# Autodesk Inventor assembly: DIFF_HOUSING_FINAL_ASM
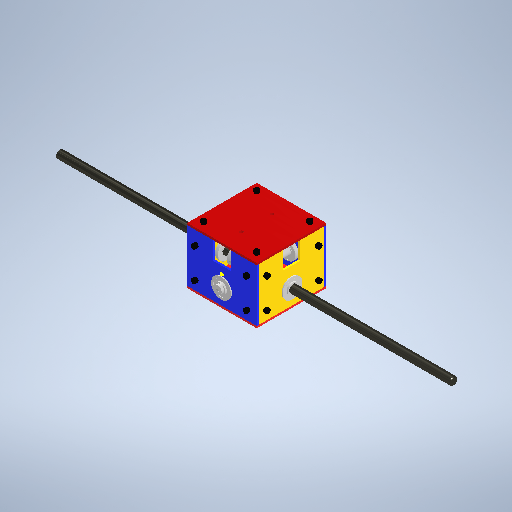
[picture p0: Inventor's stored thumbnail of the model, 512x512]
Saved by Autodesk Inventor 2025.1 (Build 291241000, 241)
## iProperties
Created: 2023-11-30
Part Number: DIFF_HOUSING_FINAL_ASM
Document SubType Name: Assembly
Designer: bugme
Author: bugme
## Documents named in this file (10)
- C:\Users\bugme\OneDrive - The Pennsylvania State University\Documents\GitHub\BehrendURCMechanical\CAD\Chassis V3\Differential Box\DIFF_HOUSING_FINAL_ASM.iam
- C:\Users\bugme\OneDrive - The Pennsylvania State University\Documents\GitHub\BehrendURCMechanical\CAD\Chassis V3\Differential Box\DIFF_HOUSING_TOP.ipt
- C:\Users\bugme\OneDrive - The Pennsylvania State University\Documents\GitHub\BehrendURCMechanical\CAD\Chassis V3\Differential Box\DIFF_PLATE_ROD.ipt
- C:\Users\bugme\OneDrive - The Pennsylvania State University\Documents\GitHub\BehrendURCMechanical\CAD\Chassis V3\Differential Box\DIFF_PLATE_ROD_SHORT.ipt
- C:\Users\bugme\OneDrive - The Pennsylvania State University\Documents\GitHub\BehrendURCMechanical\CAD\Chassis V3\Differential Box\20x20 Channel 3.33 in.ipt
- C:\Users\bugme\OneDrive - The Pennsylvania State University\Documents\GitHub\BehrendURCMechanical\CAD\Chassis V3\Differential Box\1886K21_Rotary Shaft (1)\1886K21_Rotary Shaft (1).ipt
- C:\Users\bugme\OneDrive - The Pennsylvania State University\Documents\GitHub\BehrendURCMechanical\CAD\Chassis V3\Differential Box\6529K15_Metal Miter Gear (2)\6529K15_Metal Miter Gear (2).ipt
- C:\Users\bugme\OneDrive - The Pennsylvania State University\Documents\GitHub\BehrendURCMechanical\CAD\Chassis V3\Differential Box\6384K361_Ball Bearing\6384K361_Ball Bearing.ipt
- C:\Users\bugme\OneDrive - The Pennsylvania State University\Documents\GitHub\BehrendURCMechanical\CAD\Chassis V3\Differential Box\1886K21_Rotary Shaft (1)\1886K21_Rotary Shaft _Short.ipt
- C:\Users\bugme\OneDrive - The Pennsylvania State University\Documents\GitHub\BehrendURCMechanical\CAD\Chassis V3\Differential Box\91251A342_Black-Oxide Alloy Steel Socket Head Screw\91251A342_Black-Oxide Alloy .ipt
## Components (44 placed, 9 different names)
1. DIFF_HOUSING_TOP:1 — Mate:1, Flush:2, Flush:3, Mate:2, Flush:4, Flush:5, Mate:3, Flush:6, Mate:6, Insert:1, Insert:2, Insert:3, Insert:4, Insert:31, Insert:32, Insert:33, Insert:34
2. DIFF_PLATE_ROD:1 — Mate:1, Flush:2, Flush:5, Mate:4, Mate:7, Insert:5, Insert:15, Insert:16, Insert:17, Insert:18
3. DIFF_PLATE_ROD:3 — Flush:3, Mate:2, Flush:4, Mate:5, Flush:7, Mate:9, Insert:8, Insert:23, Insert:24, Insert:25, Insert:26
4. DIFF_PLATE_ROD_SHORT:1 — Mate:3, Mate:4, Flush:6, Mate:10, Insert:6, Insert:19, Insert:20, Insert:21, Insert:22
5. DIFF_PLATE_ROD_SHORT:2 — Mate:5, Flush:7, Mate:6, Mate:8, Insert:7, Insert:27, Insert:28, Insert:29, Insert:30
6. 20x20 Channel 3.33 in:3 — Insert:1, Mate:7, Insert:9
7. 20x20 Channel 3.33 in:4 — Insert:2, Mate:8
8. 20x20 Channel 3.33 in:5 — Mate:9, Insert:3, Insert:10
9. 20x20 Channel 3.33 in:6 — Insert:4, Mate:10
10. 1886K21_Rotary Shaft (1):1 — Mate:11, Mate:12, Mate:16, Mate:18, Mate:19
11. 1886K21_Rotary Shaft (1):2 — Mate:13, Mate:14, Mate:17, Mate:20
12. 6529K15_Metal Miter Gear (2):1 — Mate:17, Mate:20
13. 6529K15_Metal Miter Gear (2):2 — Mate:18, Mate:19
14. 6529K15_Metal Miter Gear (2):3 — Mate:15, Mate:16
15. 6384K361_Ball Bearing:1 — Insert:7, Mate:13
16. 6384K361_Ball Bearing:2 — Insert:6, Mate:12
17. 6384K361_Ball Bearing:3 — Insert:5
18. 6384K361_Ball Bearing:4 — Insert:8, Cylindrical:1, Flush:8
19. 1886K21_Rotary Shaft _Short:1 — Cylindrical:1, Flush:8, Mate:11, Mate:14, Mate:15
20. DIFF_HOUSING_TOP:2 — Insert:9, Insert:10, Insert:11, Insert:12, Insert:13, Insert:14
21. 91251A342_Black-Oxide Alloy :3 — Insert:11
22. 91251A342_Black-Oxide Alloy :4 — Insert:14
23. 91251A342_Black-Oxide Alloy :5 — Insert:17
24. 91251A342_Black-Oxide Alloy :6 — Insert:18
25. 91251A342_Black-Oxide Alloy :7 — Insert:13
26. 91251A342_Black-Oxide Alloy :8 — Insert:16
27. 91251A342_Black-Oxide Alloy :9 — Insert:23
28. 91251A342_Black-Oxide Alloy :10 — Insert:22
29. 91251A342_Black-Oxide Alloy :11 — Insert:15
30. 91251A342_Black-Oxide Alloy :12 — Insert:12
31. 91251A342_Black-Oxide Alloy :13 — Insert:30
32. 91251A342_Black-Oxide Alloy :14 — Insert:25
33. 91251A342_Black-Oxide Alloy :15 — Insert:26
34. 91251A342_Black-Oxide Alloy :18 — Insert:28
35. 91251A342_Black-Oxide Alloy :19 — Insert:27
36. 91251A342_Black-Oxide Alloy :20 — Insert:19
37. 91251A342_Black-Oxide Alloy :21 — Insert:20
38. 91251A342_Black-Oxide Alloy :22 — Insert:24
39. 91251A342_Black-Oxide Alloy :23 — Insert:29
40. 91251A342_Black-Oxide Alloy :24 — Insert:21
41. 91251A342_Black-Oxide Alloy :25 — Insert:32
42. 91251A342_Black-Oxide Alloy :26 — Insert:34
43. 91251A342_Black-Oxide Alloy :27 — Insert:33
44. 91251A342_Black-Oxide Alloy :28 — Insert:31
## Relationships (62: Insert 34, Mate 20, Flush 7, CylindricalJoint 1)
- Mate:1: DIFF_HOUSING_TOP:1 ↔ DIFF_PLATE_ROD:1
- Flush:2: DIFF_HOUSING_TOP:1 ↔ DIFF_PLATE_ROD:1
- Flush:3: DIFF_HOUSING_TOP:1 ↔ DIFF_PLATE_ROD:3
- Mate:2: DIFF_HOUSING_TOP:1 ↔ DIFF_PLATE_ROD:3
- Flush:4: DIFF_HOUSING_TOP:1 ↔ DIFF_PLATE_ROD:3
- Flush:5: DIFF_HOUSING_TOP:1 ↔ DIFF_PLATE_ROD:1
- Mate:3: DIFF_HOUSING_TOP:1 ↔ DIFF_PLATE_ROD_SHORT:1
- Mate:4: DIFF_PLATE_ROD:1 ↔ DIFF_PLATE_ROD_SHORT:1
- Flush:6: DIFF_HOUSING_TOP:1 ↔ DIFF_PLATE_ROD_SHORT:1
- Mate:5: DIFF_PLATE_ROD:3 ↔ DIFF_PLATE_ROD_SHORT:2
- Flush:7: DIFF_PLATE_ROD:3 ↔ DIFF_PLATE_ROD_SHORT:2
- Mate:6: DIFF_HOUSING_TOP:1 ↔ DIFF_PLATE_ROD_SHORT:2
- Insert:1: DIFF_HOUSING_TOP:1 ↔ 20x20 Channel 3.33 in:3
- Mate:7: DIFF_PLATE_ROD:1 ↔ 20x20 Channel 3.33 in:3
- Insert:2: DIFF_HOUSING_TOP:1 ↔ 20x20 Channel 3.33 in:4
- Mate:8: DIFF_PLATE_ROD_SHORT:2 ↔ 20x20 Channel 3.33 in:4
- Mate:9: DIFF_PLATE_ROD:3 ↔ 20x20 Channel 3.33 in:5
- Insert:3: DIFF_HOUSING_TOP:1 ↔ 20x20 Channel 3.33 in:5
- Insert:4: DIFF_HOUSING_TOP:1 ↔ 20x20 Channel 3.33 in:6
- Mate:10: DIFF_PLATE_ROD_SHORT:1 ↔ 20x20 Channel 3.33 in:6
- Insert:5: DIFF_PLATE_ROD:1 ↔ 6384K361_Ball Bearing:3
- Insert:6: DIFF_PLATE_ROD_SHORT:1 ↔ 6384K361_Ball Bearing:2
- Insert:7: DIFF_PLATE_ROD_SHORT:2 ↔ 6384K361_Ball Bearing:1
- Insert:8: DIFF_PLATE_ROD:3 ↔ 6384K361_Ball Bearing:4
- Cylindrical:1: 6384K361_Ball Bearing:4 ↔ 1886K21_Rotary Shaft _Short:1
- Flush:8: 6384K361_Ball Bearing:4 ↔ 1886K21_Rotary Shaft _Short:1
- Mate:11 (12.7 mm): 1886K21_Rotary Shaft (1):1 ↔ 1886K21_Rotary Shaft _Short:1
- Mate:12: 1886K21_Rotary Shaft (1):1 ↔ 6384K361_Ball Bearing:2
- Mate:13: 1886K21_Rotary Shaft (1):2 ↔ 6384K361_Ball Bearing:1
- Mate:14 (12.7 mm): 1886K21_Rotary Shaft (1):2 ↔ 1886K21_Rotary Shaft _Short:1
- Mate:15: 6529K15_Metal Miter Gear (2):3 ↔ 1886K21_Rotary Shaft _Short:1
- Mate:16 (12.7 mm): 1886K21_Rotary Shaft (1):1 ↔ 6529K15_Metal Miter Gear (2):3
- Mate:17: 1886K21_Rotary Shaft (1):2 ↔ 6529K15_Metal Miter Gear (2):1
- Mate:18: 1886K21_Rotary Shaft (1):1 ↔ 6529K15_Metal Miter Gear (2):2
- Mate:19: 1886K21_Rotary Shaft (1):1 ↔ 6529K15_Metal Miter Gear (2):2
- Mate:20: 1886K21_Rotary Shaft (1):2 ↔ 6529K15_Metal Miter Gear (2):1
- Insert:9: 20x20 Channel 3.33 in:3 ↔ DIFF_HOUSING_TOP:2
- Insert:10: 20x20 Channel 3.33 in:5 ↔ DIFF_HOUSING_TOP:2
- Insert:11: DIFF_HOUSING_TOP:2 ↔ 91251A342_Black-Oxide Alloy :3
- Insert:12: DIFF_HOUSING_TOP:2 ↔ 91251A342_Black-Oxide Alloy :12
- Insert:13: DIFF_HOUSING_TOP:2 ↔ 91251A342_Black-Oxide Alloy :7
- Insert:14: DIFF_HOUSING_TOP:2 ↔ 91251A342_Black-Oxide Alloy :4
- Insert:15: DIFF_PLATE_ROD:1 ↔ 91251A342_Black-Oxide Alloy :11
- Insert:16: DIFF_PLATE_ROD:1 ↔ 91251A342_Black-Oxide Alloy :8
- Insert:17: DIFF_PLATE_ROD:1 ↔ 91251A342_Black-Oxide Alloy :5
- Insert:18: DIFF_PLATE_ROD:1 ↔ 91251A342_Black-Oxide Alloy :6
- Insert:19: DIFF_PLATE_ROD_SHORT:1 ↔ 91251A342_Black-Oxide Alloy :20
- Insert:20: DIFF_PLATE_ROD_SHORT:1 ↔ 91251A342_Black-Oxide Alloy :21
- Insert:21: DIFF_PLATE_ROD_SHORT:1 ↔ 91251A342_Black-Oxide Alloy :24
- Insert:22: DIFF_PLATE_ROD_SHORT:1 ↔ 91251A342_Black-Oxide Alloy :10
- Insert:23: DIFF_PLATE_ROD:3 ↔ 91251A342_Black-Oxide Alloy :9
- Insert:24: DIFF_PLATE_ROD:3 ↔ 91251A342_Black-Oxide Alloy :22
- Insert:25: DIFF_PLATE_ROD:3 ↔ 91251A342_Black-Oxide Alloy :14
- Insert:26: DIFF_PLATE_ROD:3 ↔ 91251A342_Black-Oxide Alloy :15
- Insert:27: DIFF_PLATE_ROD_SHORT:2 ↔ 91251A342_Black-Oxide Alloy :19
- Insert:28: DIFF_PLATE_ROD_SHORT:2 ↔ 91251A342_Black-Oxide Alloy :18
- Insert:29: DIFF_PLATE_ROD_SHORT:2 ↔ 91251A342_Black-Oxide Alloy :23
- Insert:30: DIFF_PLATE_ROD_SHORT:2 ↔ 91251A342_Black-Oxide Alloy :13
- Insert:31: DIFF_HOUSING_TOP:1 ↔ 91251A342_Black-Oxide Alloy :28
- Insert:32: DIFF_HOUSING_TOP:1 ↔ 91251A342_Black-Oxide Alloy :25
- Insert:33: DIFF_HOUSING_TOP:1 ↔ 91251A342_Black-Oxide Alloy :27
- Insert:34: DIFF_HOUSING_TOP:1 ↔ 91251A342_Black-Oxide Alloy :26
